# Autodesk Inventor assembly: Bended shaft concept
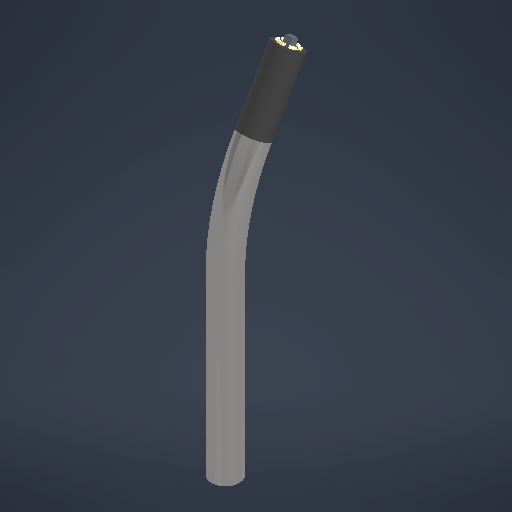
[picture p0: Inventor's stored thumbnail of the model, 512x512]
Saved by Autodesk Inventor 2026.2 (Build 302298010, 298A)
## iProperties
Created: 2026-03-31
Part Number: Bended shaft concept
Document SubType Name: Assembly
Designer: piete
Author: piete
## Documents named in this file (5)
- C:\Users\piete\Desktop\Skripsie\Documents\Concept Designs\Concept 1 Bended shaft design\Bended shaft concept.iam
- C:\Users\piete\Desktop\Skripsie\Documents\Concept Designs\Concept 1 Bended shaft design\Bended shaft.ipt
- C:\Users\piete\Desktop\Skripsie\Documents\Concept Designs\Concept 1 Bended shaft design\Camera circuit board encasing.ipt
- C:\Users\piete\Desktop\Skripsie\Documents\Concept Designs\Camera sensor.ipt
- C:\Users\piete\Desktop\Skripsie\Documents\Concept Designs\Small light.ipt
## Components (9 placed, 4 different names)
1. Bended shaft:1 — Mate:1, Mate:2, Insert:1
2. Camera circuit board encasing:1 — Mate:1, Mate:2, Insert:1, Mate:3, Mate:4, Mate:5, Mate:6, Mate:7, Mate:8, Mate:9, Mate:10, Mate:11, Mate:12, Mate:13, Angle:1, Mate:14, Mate:15, Mate:16, Mate:17, Angle:2, Mate:18, Mate:19, Angle:3, Mate:20, Mate:21, Angle:4, Mate:22, Mate:23
3. Camera sensor:1 — Mate:3, Mate:4, Mate:5
4. Small light:1 — Mate:8, Angle:1, Mate:14, Mate:16
5. Small light:2 — Mate:7, Mate:13, Mate:15
6. Small light:3 — Mate:6, Mate:12, Mate:19
7. Small light:4 — Mate:9, Mate:17, Angle:2, Mate:18
8. Small light:5 — Mate:10, Angle:3, Mate:20, Mate:21
9. Small light:6 — Mate:11, Angle:4, Mate:22, Mate:23
## Relationships (28: Mate 23, Angle 4, Insert 1)
- Mate:1: Bended shaft:1 ↔ Camera circuit board encasing:1
- Mate:2: Bended shaft:1 ↔ Camera circuit board encasing:1
- Insert:1: Bended shaft:1 ↔ Camera circuit board encasing:1
- Mate:3: Camera circuit board encasing:1 ↔ Camera sensor:1
- Mate:4: Camera circuit board encasing:1 ↔ Camera sensor:1
- Mate:5: Camera circuit board encasing:1 ↔ Camera sensor:1
- Mate:6: Camera circuit board encasing:1 ↔ Small light:3
- Mate:7: Camera circuit board encasing:1 ↔ Small light:2
- Mate:8: Camera circuit board encasing:1 ↔ Small light:1
- Mate:9: Camera circuit board encasing:1 ↔ Small light:4
- Mate:10: Camera circuit board encasing:1 ↔ Small light:5
- Mate:11: Camera circuit board encasing:1 ↔ Small light:6
- Mate:12: Camera circuit board encasing:1 ↔ Small light:3
- Mate:13: Camera circuit board encasing:1 ↔ Small light:2
- Angle:1 (-30 deg): Camera circuit board encasing:1 ↔ Small light:1
- Mate:14 (2.5 mm): Camera circuit board encasing:1 ↔ Small light:1
- Mate:15 (2.5 mm): Camera circuit board encasing:1 ↔ Small light:2
- Mate:16: Camera circuit board encasing:1 ↔ Small light:1
- Mate:17 (2.5 mm): Camera circuit board encasing:1 ↔ Small light:4
- Angle:2 (60 deg): Camera circuit board encasing:1 ↔ Small light:4
- Mate:18: Camera circuit board encasing:1 ↔ Small light:4
- Mate:19 (-2.5 mm): Camera circuit board encasing:1 ↔ Small light:3
- Angle:3 (30 deg): Camera circuit board encasing:1 ↔ Small light:5
- Mate:20 (-2.5 mm): Camera circuit board encasing:1 ↔ Small light:5
- Mate:21: Camera circuit board encasing:1 ↔ Small light:5
- Angle:4 (-60 deg): Camera circuit board encasing:1 ↔ Small light:6
- Mate:22 (-2.5 mm): Camera circuit board encasing:1 ↔ Small light:6
- Mate:23: Camera circuit board encasing:1 ↔ Small light:6
